# Autodesk Inventor assembly: Rail assembly
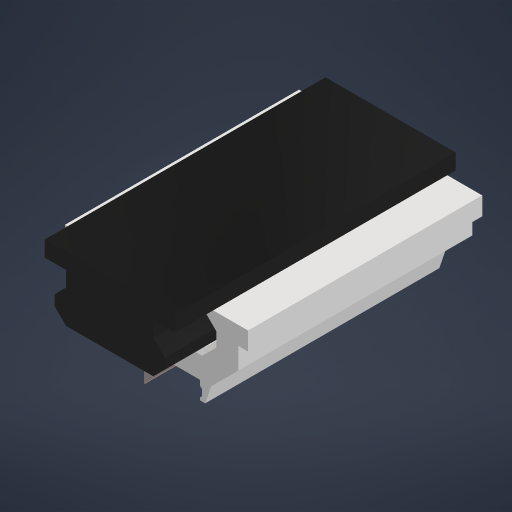
[picture p0: Inventor's stored thumbnail of the model, 512x512]
Saved by Autodesk Inventor 2023 (Build 270158000, 158)
## iProperties
Created: 2023-10-16
Part Number: Rail assembly
Document SubType Name: Assembly
Designer: nick_
Author: nick_
## Documents named in this file (4)
- D:\Github\Classpert_GreenTurtles\Final project\Mechanical\Rail assembly.iam
- D:\Github\Classpert_GreenTurtles\Final project\Mechanical\Rail\Picatinny model.ipt
- D:\Github\Classpert_GreenTurtles\Final project\Mechanical\Rail clamp.ipt
- D:\Github\Classpert_GreenTurtles\Final project\Mechanical\IMU Module.ipt
## Components (3 placed, 3 different names)
1. Picatinny model:1 — Flush:1
2. Rail clamp:1 — Flush:1, Mate:1, Mate:2
3. IMU Module:1 — Mate:1, Mate:2
## Relationships (3: Mate 2, Flush 1)
- Flush:1: Picatinny model:1 ↔ Rail clamp:1
- Mate:1 (1.2 mm): Rail clamp:1 ↔ IMU Module:1
- Mate:2 (1.947 mm): Rail clamp:1 ↔ IMU Module:1
